# Autodesk Inventor assembly: rays demo
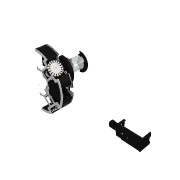
[picture p0: Inventor's stored thumbnail of the model, 180x180]
Saved by Autodesk Inventor 2020 (Build 240168000, 168)
## iProperties
Created: 2024-02-27
Part Number: rays demo
Document SubType Name: Assembly
Designer: 4s
Author: 4s
## Documents named in this file (3)
- C:\Users\4s\Documents\Inventor models\Asterisk\robot_v2\rays demo.iam
- C:\Users\4s\Documents\Inventor models\Asterisk\Free models\field.ipt
- C:\Users\4s\Documents\Inventor models\Asterisk\robot_v2\main2.iam
## Components (2 placed, 2 different names)
1. field:1 — Заподлицо:1, Совмещение:1, Заподлицо:2, Совмещение:2, Совмещение:4, Угол:1, Совмещение:5, Заподлицо:3
2. main2:2 [sub-assembly] — Совмещение:4, Угол:1, Совмещение:5
## Relationships (8: Mate 4, Flush 3, Angle 1)
- Заподлицо:1 [Flush]: field:1
- Совмещение:1 [Mate]: field:1
- Заподлицо:2 [Flush]: field:1
- Совмещение:2 [Mate]: field:1
- Совмещение:4 [Mate] (9 mm): field:1 ↔ main2:2
- Угол:1 [Angle] (90 deg): field:1 ↔ main2:2
- Совмещение:5 [Mate]: field:1 ↔ main2:2
- Заподлицо:3 [Flush] (910 mm): field:1
